# Autodesk Inventor assembly: захват спереди
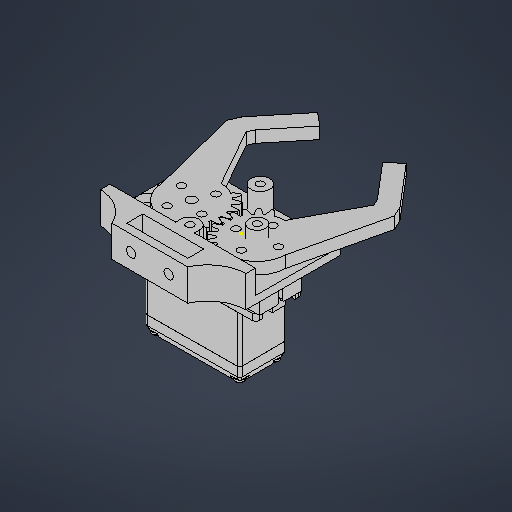
[picture p0: Inventor's stored thumbnail of the model, 512x512]
Saved by Autodesk Inventor 2025 (Build 290162000, 162)
## iProperties
Created: 2025-02-22
Part Number: захват спереди
Document SubType Name: Assembly
Designer: Phantom
Author: Phantom
## Documents named in this file (6)
- C:\Users\Phantom\Desktop\Phantom16950\захват спереди.iam
- C:\Users\Phantom\Desktop\Phantom16950\крышка захвата.ipt
- C:\Users\Phantom\Desktop\Phantom16950\ПЕРЕДНИЙ ЗАХВАТ.ipt
- C:\Users\Phantom\Desktop\Phantom16950\2000-0025-0002\2000-0025-0002_MIR2_MIR1.ipt
- C:\Users\Phantom\Desktop\Phantom16950\писюн 2.ipt
- C:\Users\Phantom\Desktop\Phantom16950\писюн.ipt
## Components (5 placed, 5 different names)
1. крышка захвата:1 — Совмещение:1, Совмещение:14, Совмещение:15
2. ПЕРЕДНИЙ ЗАХВАТ:1 — Совмещение:1, Совмещение:7, Совмещение:8, Совмещение:10, Совмещение:11, Совмещение:12, Совмещение:13, Совмещение:14, Совмещение:15
3. 2000-0025-0002_MIR2_MIR1:1 — Совмещение:7, Совмещение:8
4. писюн 2:1 — Совмещение:10, Совмещение:11
5. писюн:1 — Совмещение:12, Совмещение:13
## Relationships (9: Mate 9)
- Совмещение:1 [Mate]: крышка захвата:1 ↔ ПЕРЕДНИЙ ЗАХВАТ:1
- Совмещение:7 [Mate]: ПЕРЕДНИЙ ЗАХВАТ:1 ↔ 2000-0025-0002_MIR2_MIR1:1
- Совмещение:8 [Mate]: ПЕРЕДНИЙ ЗАХВАТ:1 ↔ 2000-0025-0002_MIR2_MIR1:1
- Совмещение:10 [Mate]: ПЕРЕДНИЙ ЗАХВАТ:1 ↔ писюн 2:1
- Совмещение:11 [Mate]: ПЕРЕДНИЙ ЗАХВАТ:1 ↔ писюн 2:1
- Совмещение:12 [Mate]: ПЕРЕДНИЙ ЗАХВАТ:1 ↔ писюн:1
- Совмещение:13 [Mate]: ПЕРЕДНИЙ ЗАХВАТ:1 ↔ писюн:1
- Совмещение:14 [Mate]: крышка захвата:1 ↔ ПЕРЕДНИЙ ЗАХВАТ:1
- Совмещение:15 [Mate]: крышка захвата:1 ↔ ПЕРЕДНИЙ ЗАХВАТ:1
